# Autodesk Inventor assembly: Ball Shooter Wheel Sub-Assembly V2
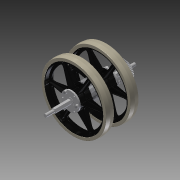
[picture p0: Inventor's stored thumbnail of the model, 180x180]
Saved by Autodesk Inventor 2014 SP1 (Build 180222100, 222)
## iProperties
Created: 2012-01-30
Part Number: Ball Shooter Wheel Sub-Assembly V2
Document SubType Name: Assembly
Designer: Moses
Mass: 1114.7 g
Surface Area: 3411.87 cm^2
Volume: 718.56 cm^3
Density: 1.55129 g/cm^3
Author: Moses
## Documents named in this file (9)
- C:\Users\Moses\Documents\GitHub\frc2014CAD\2012\Repackaged_Team_3061_Yr2012_Ball_Shooter\Ball Shooter Wheel Sub-Assembly V2.iam
- C:\Users\Moses\Documents\GitHub\frc2014CAD\2012\Repackaged_Team_3061_Yr2012_Ball_Shooter\8-inch-FIRST-Wheel.iam
- C:\Users\Moses\Documents\GitHub\frc2014CAD\2012\Repackaged_Team_3061_Yr2012_Ball_Shooter\Custom Hex Hub.ipt
- C:\Users\Moses\Documents\GitHub\frc2014CAD\2012\Repackaged_Team_3061_Yr2012_Ball_Shooter\Spacer Between Wheels V2.ipt
- C:\Users\Moses\Documents\GitHub\frc2014CAD\2012\Repackaged_Team_3061_Yr2012_Ball_Shooter\AM-0129 Large Final Gear 45T.ipt
- C:\Users\Moses\Documents\GitHub\frc2014CAD\2012\Repackaged_Team_3061_Yr2012_Ball_Shooter\0.5 in Hex Shaft V3.ipt
- C:\Users\Moses\Documents\GitHub\frc2014CAD\2012\Repackaged_Team_3061_Yr2012_Ball_Shooter\ANSI B27.7M - 3CMI-15.ipt
- C:\Users\Moses\Documents\GitHub\frc2014CAD\2012\Repackaged_Team_3061_Yr2012_Ball_Shooter\Threaded Rod.ipt
- C:\Users\Moses\Documents\GitHub\frc2014CAD\2012\Repackaged_Team_3061_Yr2012_Ball_Shooter\Nut GB_T 41 M5.ipt
## Components (20 placed, 8 different names)
1. 8-inch-FIRST-Wheel:1 [sub-assembly] — Insert:1, Mate:2, Insert:4, Mate:4
2. 8-inch-FIRST-Wheel:2 [sub-assembly] — Insert:2, Mate:1, Insert:5, Mate:6
3. Custom Hex Hub:1 — Insert:1, Mate:2, Mate:19, Mate:20, Mate:21, Flush:3, Flush:4, Flush:5, Insert:6, Insert:7, Insert:8
4. Custom Hex Hub:2 — Insert:2, Mate:1, Mate:9, Mate:10, Flush:2, Insert:9, Insert:10, Insert:11
5. Spacer Between Wheels V2:1 — Insert:4, Mate:4, Insert:5, Mate:6
6. AM-0129 Large Final Gear 45T:1 — Mate:7, Mate:8, Flush:1
7. 0.5 in Hex Shaft V3:1 — Mate:7, Mate:8, Mate:9, Mate:10, Flush:1, Flush:2, Mate:11, Mate:12, Mate:13, Mate:14, Mate:15, Mate:16, Mate:17, Mate:18
8. ANSI B27.7M 3CMI-15:1 — Mate:11, Mate:12
9. ANSI B27.7M 3CMI-15:2 — Mate:13, Mate:14
10. ANSI B27.7M 3CMI-15:3 — Mate:15, Mate:16
11. ANSI B27.7M 3CMI-15:4 — Mate:17, Mate:18
12. Threaded Rod:1 — Mate:19, Flush:3
13. Threaded Rod:2 — Mate:20, Flush:4
14. Threaded Rod:3 — Mate:21, Flush:5
15. Nut GB/T 41-2000 M 5:1 — Insert:6
16. Nut GB/T 41-2000 M 5:2 — Insert:7
17. Nut GB/T 41-2000 M 5:3 — Insert:8
18. Nut GB/T 41-2000 M 5:4 — Insert:9
19. Nut GB/T 41-2000 M 5:5 — Insert:10
20. Nut GB/T 41-2000 M 5:6 — Insert:11
## Relationships (34: Mate 19, Insert 10, Flush 5)
- Insert:1: 8-inch-FIRST-Wheel:1 ↔ Custom Hex Hub:1
- Insert:2: 8-inch-FIRST-Wheel:2 ↔ Custom Hex Hub:2
- Mate:1: 8-inch-FIRST-Wheel:2 ↔ Custom Hex Hub:2
- Mate:2: 8-inch-FIRST-Wheel:1 ↔ Custom Hex Hub:1
- Insert:4: 8-inch-FIRST-Wheel:1 ↔ Spacer Between Wheels V2:1
- Mate:4: 8-inch-FIRST-Wheel:1 ↔ Spacer Between Wheels V2:1
- Insert:5: 8-inch-FIRST-Wheel:2 ↔ Spacer Between Wheels V2:1
- Mate:6: 8-inch-FIRST-Wheel:2 ↔ Spacer Between Wheels V2:1
- Mate:7: AM-0129 Large Final Gear 45T:1 ↔ 0.5 in Hex Shaft V3:1
- Mate:8: AM-0129 Large Final Gear 45T:1 ↔ 0.5 in Hex Shaft V3:1
- Mate:9: Custom Hex Hub:2 ↔ 0.5 in Hex Shaft V3:1
- Mate:10: Custom Hex Hub:2 ↔ 0.5 in Hex Shaft V3:1
- Flush:1: AM-0129 Large Final Gear 45T:1 ↔ 0.5 in Hex Shaft V3:1
- Flush:2: Custom Hex Hub:2 ↔ 0.5 in Hex Shaft V3:1
- Mate:12: 0.5 in Hex Shaft V3:1 ↔ ANSI B27.7M 3CMI-15:1
- Mate:14: 0.5 in Hex Shaft V3:1 ↔ ANSI B27.7M 3CMI-15:2
- Mate:16: 0.5 in Hex Shaft V3:1 ↔ ANSI B27.7M 3CMI-15:3
- Mate:18: 0.5 in Hex Shaft V3:1 ↔ ANSI B27.7M 3CMI-15:4
- Mate:19: Custom Hex Hub:1 ↔ Threaded Rod:1
- Mate:20: Custom Hex Hub:1 ↔ Threaded Rod:2
- Mate:21: Custom Hex Hub:1 ↔ Threaded Rod:3
- Flush:3 (-8.128 mm): Custom Hex Hub:1 ↔ Threaded Rod:1
- Flush:4 (-8.128 mm): Custom Hex Hub:1 ↔ Threaded Rod:2
- Flush:5 (-8.128 mm): Custom Hex Hub:1 ↔ Threaded Rod:3
- Mate:11: 0.5 in Hex Shaft V3:1 ↔ ANSI B27.7M 3CMI-15:1
- Mate:13: 0.5 in Hex Shaft V3:1 ↔ ANSI B27.7M 3CMI-15:2
- Mate:15: 0.5 in Hex Shaft V3:1 ↔ ANSI B27.7M 3CMI-15:3
- Mate:17: 0.5 in Hex Shaft V3:1 ↔ ANSI B27.7M 3CMI-15:4
- Insert:6: Custom Hex Hub:1 ↔ Nut GB/T 41-2000 M 5:1
- Insert:7: Custom Hex Hub:1 ↔ Nut GB/T 41-2000 M 5:2
- Insert:8: Custom Hex Hub:1 ↔ Nut GB/T 41-2000 M 5:3
- Insert:9: Custom Hex Hub:2 ↔ Nut GB/T 41-2000 M 5:4
- Insert:10: Custom Hex Hub:2 ↔ Nut GB/T 41-2000 M 5:5
- Insert:11: Custom Hex Hub:2 ↔ Nut GB/T 41-2000 M 5:6
